# Autodesk Inventor assembly: Pull Tester
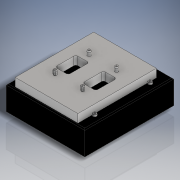
[picture p0: Inventor's stored thumbnail of the model, 180x180]
Saved by Autodesk Inventor 2019.4 (Build 234330000, 330)
## iProperties
Created: 2020-11-12
Part Number: Pull Tester
Document SubType Name: Assembly
Designer: caleb
Author: caleb
## Documents named in this file (8)
- C:\Users\cfang\Desktop\CAD\Pull Tester\Pull Tester.iam
- C:\Users\cfang\Desktop\CAD\Pull Tester\Chuck.ipt
- C:\Users\cfang\Desktop\CAD\Pull Tester\step_12692.ipt
- C:\Users\cfang\Desktop\CAD\Pull Tester\90128A211_ZNC-PLTD ALLOY STL SCKT HEAD CAP SCREW.ipt
- C:\Users\cfang\Desktop\CAD\Pull Tester\90128A263_ZNC-PLTD ALLOY STL SCKT HEAD CAP SCREW.ipt
- C:\Users\cfang\Desktop\CAD\Pull Tester\TFPX Plate.ipt
- C:\Users\cfang\Desktop\CAD\Pull Tester\8472A190_PRESS-FIT LOCATING PIN.ipt
- C:\Users\cfang\Desktop\CAD\Pull Tester\8472A110_PRESS-FIT LOCATING PIN.ipt
## Components (15 placed, 7 different names)
1. Chuck:1 — Insert:4, Insert:5, Insert:6, Insert:7, Mate:1, Mate:2, Insert:9, Insert:10, Insert:11, Insert:12, Mate:4
2. step_12692:1 — Mate:1, Mate:2
3. 90128A211_ZNC-PLTD ALLOY STL SCKT HEAD CAP SCREW:4 — Insert:4, Tangent:1
4. 90128A211_ZNC-PLTD ALLOY STL SCKT HEAD CAP SCREW:5 — Insert:5, Tangent:2
5. 90128A211_ZNC-PLTD ALLOY STL SCKT HEAD CAP SCREW:6 — Insert:6, Tangent:3
6. 90128A211_ZNC-PLTD ALLOY STL SCKT HEAD CAP SCREW:7 — Insert:7
7. 90128A263_ZNC-PLTD ALLOY STL SCKT HEAD CAP SCREW:1 — Insert:9
8. 90128A263_ZNC-PLTD ALLOY STL SCKT HEAD CAP SCREW:2 — Insert:10
9. 90128A263_ZNC-PLTD ALLOY STL SCKT HEAD CAP SCREW:3 — Insert:11
10. 90128A263_ZNC-PLTD ALLOY STL SCKT HEAD CAP SCREW:4 — Insert:12
11. TFPX Plate:1 — Mate:4, Tangent:1, Tangent:2, Tangent:3, Insert:13, Insert:14, Insert:15, Insert:16
12. 8472A190_PRESS-FIT LOCATING PIN:1 — Insert:15
13. 8472A110_PRESS-FIT LOCATING PIN:1 — Insert:14
14. 8472A110_PRESS-FIT LOCATING PIN:2 — Insert:13
15. 8472A190_PRESS-FIT LOCATING PIN:2 — Insert:16
## Relationships (18: Insert 12, Mate 3, Tangent 3)
- Insert:4: Chuck:1 ↔ 90128A211_ZNC-PLTD ALLOY STL SCKT HEAD CAP SCREW:4
- Insert:5: Chuck:1 ↔ 90128A211_ZNC-PLTD ALLOY STL SCKT HEAD CAP SCREW:5
- Insert:6: Chuck:1 ↔ 90128A211_ZNC-PLTD ALLOY STL SCKT HEAD CAP SCREW:6
- Insert:7: Chuck:1 ↔ 90128A211_ZNC-PLTD ALLOY STL SCKT HEAD CAP SCREW:7
- Mate:1: Chuck:1 ↔ step_12692:1
- Mate:2: Chuck:1 ↔ step_12692:1
- Insert:9: Chuck:1 ↔ 90128A263_ZNC-PLTD ALLOY STL SCKT HEAD CAP SCREW:1
- Insert:10: Chuck:1 ↔ 90128A263_ZNC-PLTD ALLOY STL SCKT HEAD CAP SCREW:2
- Insert:11: Chuck:1 ↔ 90128A263_ZNC-PLTD ALLOY STL SCKT HEAD CAP SCREW:3
- Insert:12: Chuck:1 ↔ 90128A263_ZNC-PLTD ALLOY STL SCKT HEAD CAP SCREW:4
- Mate:4: Chuck:1 ↔ TFPX Plate:1
- Tangent:1: 90128A211_ZNC-PLTD ALLOY STL SCKT HEAD CAP SCREW:4 ↔ TFPX Plate:1
- Tangent:2: 90128A211_ZNC-PLTD ALLOY STL SCKT HEAD CAP SCREW:5 ↔ TFPX Plate:1
- Tangent:3: 90128A211_ZNC-PLTD ALLOY STL SCKT HEAD CAP SCREW:6 ↔ TFPX Plate:1
- Insert:13: TFPX Plate:1 ↔ 8472A110_PRESS-FIT LOCATING PIN:2
- Insert:14: TFPX Plate:1 ↔ 8472A110_PRESS-FIT LOCATING PIN:1
- Insert:15: TFPX Plate:1 ↔ 8472A190_PRESS-FIT LOCATING PIN:1
- Insert:16: TFPX Plate:1 ↔ 8472A190_PRESS-FIT LOCATING PIN:2
